# Autodesk Inventor assembly: Мостики
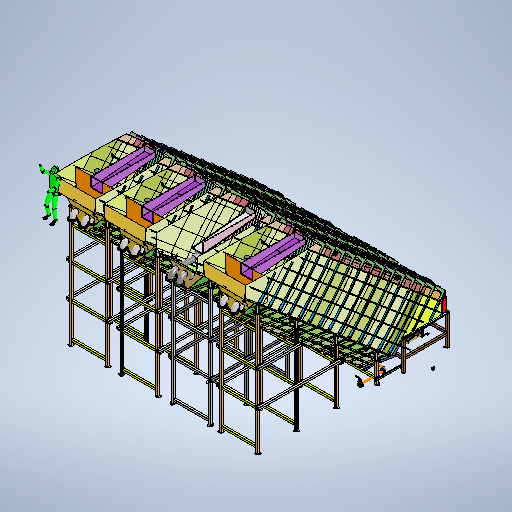
[picture p0: Inventor's stored thumbnail of the model, 512x512]
Saved by Autodesk Inventor 2025 (Build 290162010, 162A)
## iProperties
Created: 2025-01-27
Part Number: Мостики
Document SubType Name: Assembly
Designer: admin
Author: admin
## Documents named in this file (4)
- C:\Users\admin\YandexDisk-badmisterfox\домашниий пк\Inventor\Manturovo\Manturovo_Se-clar\Мостики.iam
- C:\Users\admin\YandexDisk-badmisterfox\домашниий пк\Inventor\Manturovo\Manturovo_Se-clar\ASY MSC 002 отстойник осветлитель.iam
- C:\Users\admin\YandexDisk-badmisterfox\домашниий пк\Inventor\Manturovo\АРХИВНЫЙ Manturovo_Se-clar\ASY MSC 001 АРХИВ отстойник осветлитель.iam
- C:\Users\admin\YandexDisk-badmisterfox\домашниий пк\Inventor\Manturovo\Manturovo_Se-clar\human 01\ч ASY human dummy 01.iam
## Components (5 placed, 3 different names)
1. ASY MSC 002 отстойник осветлитель:1 [sub-assembly] — Flush:1
2. ASY MSC 002 отстойник осветлитель:2 [sub-assembly]
3. ASY MSC 002 отстойник осветлитель:3 [sub-assembly]
4. ASY MSC 001 АРХИВ отстойник осветлитель:1 [sub-assembly]
5. ч ASY human dummy 01:1 [sub-assembly] — Flush:1
## Relationships (1: Flush 1)
- Flush:1 (4500 mm): ASY MSC 002 отстойник осветлитель:1 ↔ ч ASY human dummy 01:1
